# Autodesk Inventor assembly: SFU1605KIT
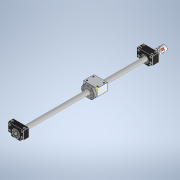
[picture p0: Inventor's stored thumbnail of the model, 180x180]
Saved by Autodesk Inventor 2022 (Build 260153000, 153)
## iProperties
Created: 2019-09-26
Part Number: SFU1605KIT
Document SubType Name: Assembly
Designer: JK
Sending System: Autodesk Translation Framework v8.6.0.1094
Preprocessor: ST-DEVELOPER v18
Title: D:/3DPrinter/CoreXY/Ball Screw Kit/1605 Ball Screw Kit .step
## Documents named in this file (7)
- C:\Users\JK\Documents\Inventor\UTM\SFU1605KIT.iam
- C:\Users\JK\Documents\Inventor\UTM\BK Block.iam
- C:\Users\JK\Documents\Inventor\UTM\BF Block.iam
- C:\Users\JK\Documents\Inventor\UTM\Carriage.iam
- C:\Users\JK\Documents\Inventor\UTM\LEADBALLSCREW1605.ipt
- C:\Users\JK\Documents\Inventor\UTM\NutCarriage.ipt
- C:\Users\JK\Documents\Inventor\UTM\Flexcoupling8-10.ipt
## Components (6 placed, 6 different names)
1. BK Block:1 [sub-assembly] — Coincidencia:11, Coincidencia:12, Ángulo:2, Ángulo:3
2. BF Block:1 [sub-assembly] — Coincidencia:9, Coincidencia:10, Ángulo:2
3. Carriage:1 [sub-assembly] — Coincidencia:1, Coincidencia:6, Ángulo:1, Coincidencia:7
4. LEADBALLSCREW1605:1 — Coincidencia:1, Coincidencia:9, Coincidencia:10, Coincidencia:11, Coincidencia:12, Coincidencia:13, Coincidencia:14
5. NutCarriage:1 — Coincidencia:6, Ángulo:1, Coincidencia:7, Ángulo:3
6. Flexcoupling8-10:1 — Coincidencia:13, Coincidencia:14
## Relationships (12: Mate 9, Angle 3)
- Coincidencia:1 [Mate]: Carriage:1 ↔ LEADBALLSCREW1605:1
- Coincidencia:6 [Mate]: Carriage:1 ↔ NutCarriage:1
- Ángulo:1 [Angle] (0 deg): Carriage:1 ↔ NutCarriage:1
- Coincidencia:7 [Mate]: Carriage:1 ↔ NutCarriage:1
- Coincidencia:9 [Mate]: BF Block:1 ↔ LEADBALLSCREW1605:1
- Coincidencia:10 [Mate]: BF Block:1 ↔ LEADBALLSCREW1605:1
- Coincidencia:11 [Mate]: BK Block:1 ↔ LEADBALLSCREW1605:1
- Coincidencia:12 [Mate]: BK Block:1 ↔ LEADBALLSCREW1605:1
- Ángulo:2 [Angle] (0 deg): BK Block:1 ↔ BF Block:1
- Coincidencia:13 [Mate]: LEADBALLSCREW1605:1 ↔ Flexcoupling8-10:1
- Coincidencia:14 [Mate]: LEADBALLSCREW1605:1 ↔ Flexcoupling8-10:1
- Ángulo:3 [Angle] (0 deg): BK Block:1 ↔ NutCarriage:1
